# Autodesk Inventor assembly: Drinkmixer.Rohr- und Leitungsverläufe01
(part 2 of 2)
## Documents named in this file (2)
- D:\Dropbox\My Dropbox\Dokumente\Aktuell\Drinkmixer\Drinkmixer\AIP\Rohr und Leitung\Drinkmixer.Rohr- und Leitungsverläufe01.iam
- D:\Dropbox\My Dropbox\Dokumente\Aktuell\Drinkmixer\Drinkmixer\AIP\Rohr und Leitung\Verlauf02\Drinkmixer.Verlauf02.iam
## Components (1 placed, 1 different names)
1. Verlauf02 [sub-assembly]
